# Autodesk Inventor assembly: Heating Plate
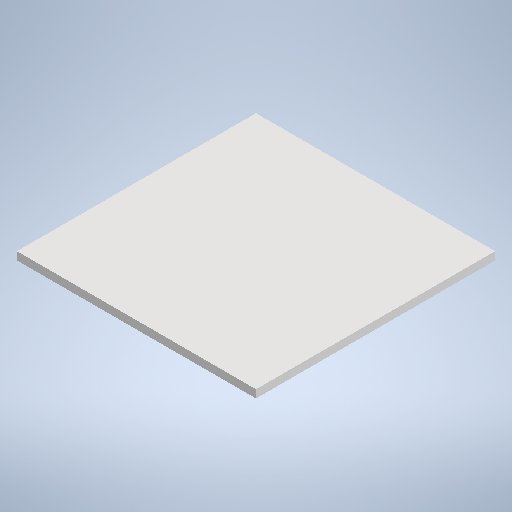
[picture p0: Inventor's stored thumbnail of the model, 512x512]
Saved by Autodesk Inventor 2025.1 (Build 291241020, 241B)
## iProperties
Created: 2024-10-29
Part Number: Heating Plate
Document SubType Name: Assembly
Designer: jjk
Author: jjk
## Documents named in this file (3)
- C:\Users\jjk\Desktop\Capstone CAD\Version 2\Heating Plate.iam
- C:\Users\jjk\Desktop\Capstone CAD\Version 2\Heating board.ipt
- C:\Users\jjk\Desktop\Capstone CAD\Version 2\flat 32 gauge nichrome wire.ipt
## Components (7 placed, 2 different names)
1. Heating board:1 — Mate:4, Flush:1, Flush:3, Mate:5, Flush:5, Mate:6, Flush:7, Mate:7, Flush:9, Mate:8, Flush:11, Mate:9
2. flat 32 gauge nichrome wire:2 — Mate:4, Flush:1
3. flat 32 gauge nichrome wire:1 — Flush:3, Mate:5
4. flat 32 gauge nichrome wire:3 — Flush:5, Mate:6
5. flat 32 gauge nichrome wire:4 — Flush:7, Mate:7
6. flat 32 gauge nichrome wire:5 — Flush:9, Mate:8
7. flat 32 gauge nichrome wire:6 — Flush:11, Mate:9
## Relationships (12: Mate 6, Flush 6)
- Mate:4: Heating board:1 ↔ flat 32 gauge nichrome wire:2
- Flush:1: Heating board:1 ↔ flat 32 gauge nichrome wire:2
- Flush:3: Heating board:1 ↔ flat 32 gauge nichrome wire:1
- Mate:5: Heating board:1 ↔ flat 32 gauge nichrome wire:1
- Flush:5: Heating board:1 ↔ flat 32 gauge nichrome wire:3
- Mate:6: Heating board:1 ↔ flat 32 gauge nichrome wire:3
- Flush:7: Heating board:1 ↔ flat 32 gauge nichrome wire:4
- Mate:7: Heating board:1 ↔ flat 32 gauge nichrome wire:4
- Flush:9: Heating board:1 ↔ flat 32 gauge nichrome wire:5
- Mate:8: Heating board:1 ↔ flat 32 gauge nichrome wire:5
- Flush:11: Heating board:1 ↔ flat 32 gauge nichrome wire:6
- Mate:9: Heating board:1 ↔ flat 32 gauge nichrome wire:6
## Named parameters: Finish1_Area = 232.258, Finish2_Area = 232.258
note: some values were not read from the file. Shown as the stored number, unit unknown: "Finish1_Area", "Finish2_Area".
